# Autodesk Inventor assembly: RatchetSprocket
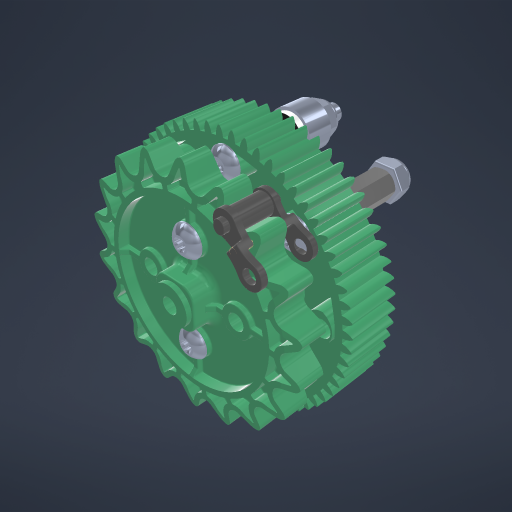
[picture p0: Inventor's stored thumbnail of the model, 512x512]
Saved by Autodesk Inventor 2023 (Build 270158000, 158)
## iProperties
Created: 2022-11-12
Part Number: RatchetSprocket
Document SubType Name: Assembly
Designer: alex
Author: alex
## Documents named in this file (19)
- C:\Users\alex\Documents\GitHub\4067X_spin_up_cad\RatchetSprocket.iam
- C:\Users\alex\Documents\GitHub\4067X_spin_up_cad\Library\Motion\Gears\HS 60T Gear, Circle.ipt
- C:\Users\alex\Documents\GitHub\4067X_spin_up_cad\Library\Motion\Sprockets\HS 6T Sprocket, Square.ipt
- C:\Users\alex\Documents\GitHub\4067X_spin_up_cad\Library\Motion\Sprockets\HS 18T Sprocket, Circle.ipt
- C:\Users\alex\Documents\GitHub\4067X_spin_up_cad\Library\Motion\Spacers\Spacer Nylon .375 OD\NSpacer .375 OD x .375.ipt
- C:\Users\alex\Documents\GitHub\4067X_spin_up_cad\Library\Motion\Spacers\Spacer Nylon .375 OD.ipt
- C:\Users\alex\Documents\GitHub\4067X_spin_up_cad\Library\Motion\Spacers\Washer Teflon\TWasher .375 OD x .03125.ipt
- C:\Users\alex\Documents\GitHub\4067X_spin_up_cad\Library\Motion\Spacers\Washer Teflon.ipt
- C:\Users\alex\Documents\GitHub\4067X_spin_up_cad\Library\Structure\Hardware\Screw Steel - Star\SScrew Star Smooth .875.ipt
- C:\Users\alex\Documents\GitHub\4067X_spin_up_cad\Library\Structure\Hardware\Screw Steel - Star.ipt
- C:\Users\alex\Documents\GitHub\4067X_spin_up_cad\Library\Structure\Hardware\Nut Thin Nylock.ipt
- C:\Users\alex\Documents\GitHub\4067X_spin_up_cad\Library\Motion\Spacers\Spacer Nylon .375 OD\NSpacer .375 OD x .125.ipt
- C:\Users\alex\Documents\GitHub\4067X_spin_up_cad\Library\Motion\Shaft Collar without Set Screw.ipt
- C:\Users\alex\Documents\GitHub\4067X_spin_up_cad\Library\Motion\Spacers\Washer Teflon\TWasher .375 OD x .06250.ipt
- C:\Users\alex\Documents\GitHub\4067X_spin_up_cad\Library\Structure\Hardware\Screw Steel - Star\SScrew Star Smooth .625.ipt
- C:\Users\alex\Documents\GitHub\4067X_spin_up_cad\Library\Structure\Hardware\Screw Steel - Star\SScrew Star Smooth 1.250.ipt
- C:\Users\alex\Documents\GitHub\4067X_spin_up_cad\Library\Structure\Standoff\Standoff .50.ipt
- C:\Users\alex\Documents\GitHub\4067X_spin_up_cad\Library\Structure\Standoff.ipt
- C:\Users\alex\Documents\GitHub\4067X_spin_up_cad\Library\Motion\Chain + Tank Tread\High Strength Chain Link.ipt
## Components (21 placed, 14 different names)
1. HS 60T Gear, Circle:1 — Insert:3, Insert:4, Insert:5, Insert:8, Insert:12, Insert:16, Insert:18, Insert:21, Insert:22
2. HS 6T Sprocket, Square:1 — Insert:8
3. HS 18T Sprocket, Circle:1 — Insert:1, Insert:2, Insert:20, Mate:3, Mate:4
4. NSpacer .375 OD x .375:1 — Insert:19, Insert:20
5. TWasher .375 OD x .03125:1 — Insert:18, Insert:19
6. TWasher .375 OD x .03125:2 — Insert:16, Insert:17
7. NSpacer .375 OD x .375:2 — Insert:17, Mate:2
8. SScrew Star Smooth .875:1 — Insert:1
9. SScrew Star Smooth .875:2 — Insert:2, Mate:2
10. Nut Thin Nylock:1 — Insert:3
11. Nut Thin Nylock:2 — Insert:4
12. NSpacer .375 OD x .125:3 — Insert:5, Insert:6
13. Shaft Collar without Set Screw:1 — Insert:7, Mate:1, Insert:11
14. TWasher .375 OD x .06250:3 — Insert:6, Insert:7
15. SScrew Star Smooth .625:3 — Mate:1
16. SScrew Star Smooth 1.250:4 — Insert:21
17. Nut Thin Nylock:3 — Insert:11
18. Standoff .50:1 — Insert:12, Insert:15
19. SScrew Star Smooth 1.250:5 — Insert:22
20. Nut Thin Nylock:4 — Insert:15
21. High Strength Chain Link:1 — Mate:3, Mate:4
## Relationships (22: Insert 18, Mate 4)
- Insert:1: HS 18T Sprocket, Circle:1 ↔ SScrew Star Smooth .875:1
- Insert:2: HS 18T Sprocket, Circle:1 ↔ SScrew Star Smooth .875:2
- Insert:3: HS 60T Gear, Circle:1 ↔ Nut Thin Nylock:1
- Insert:4: HS 60T Gear, Circle:1 ↔ Nut Thin Nylock:2
- Insert:5: HS 60T Gear, Circle:1 ↔ NSpacer .375 OD x .125:3
- Insert:6: NSpacer .375 OD x .125:3 ↔ TWasher .375 OD x .06250:3
- Insert:7: Shaft Collar without Set Screw:1 ↔ TWasher .375 OD x .06250:3
- Insert:8: HS 60T Gear, Circle:1 ↔ HS 6T Sprocket, Square:1
- Mate:1: Shaft Collar without Set Screw:1 ↔ SScrew Star Smooth .625:3
- Insert:11: Shaft Collar without Set Screw:1 ↔ Nut Thin Nylock:3
- Insert:12: HS 60T Gear, Circle:1 ↔ Standoff .50:1
- Insert:15: Standoff .50:1 ↔ Nut Thin Nylock:4
- Insert:16: HS 60T Gear, Circle:1 ↔ TWasher .375 OD x .03125:2
- Insert:17: TWasher .375 OD x .03125:2 ↔ NSpacer .375 OD x .375:2
- Insert:18: HS 60T Gear, Circle:1 ↔ TWasher .375 OD x .03125:1
- Insert:19: NSpacer .375 OD x .375:1 ↔ TWasher .375 OD x .03125:1
- Insert:20: HS 18T Sprocket, Circle:1 ↔ NSpacer .375 OD x .375:1
- Mate:2: NSpacer .375 OD x .375:2 ↔ SScrew Star Smooth .875:2
- Insert:21: HS 60T Gear, Circle:1 ↔ SScrew Star Smooth 1.250:4
- Insert:22: HS 60T Gear, Circle:1 ↔ SScrew Star Smooth 1.250:5
- Mate:3: HS 18T Sprocket, Circle:1 ↔ High Strength Chain Link:1
- Mate:4: HS 18T Sprocket, Circle:1 ↔ High Strength Chain Link:1
